# Autodesk Inventor assembly: AK-C-C39-USB-Board-Assembly
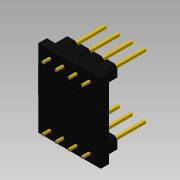
[picture p0: Inventor's stored thumbnail of the model, 180x180]
Saved by Autodesk Inventor 2016 (Build 200138000, 138)
## iProperties
Created: 2016-06-09
Part Number: AK-C-C39-USB-Board-Assembly
Document SubType Name: Assembly
Designer: admin
Author: admin
## Documents named in this file (4)
- E:\Alex\DI-Lambda\parts\v1\AK-C-C39\AK-C-C39-USB-Board-Assembly.iam
- E:\Alex\DI-Lambda\parts\v1\AK-C-C39\Ak-C-C39-USB-board.ipt
- E:\Alex\DI-Lambda\parts\Common\fciconnect-10118194.ipt
- E:\Alex\DI-Lambda\parts\Common\Pin-round-2.54-male.ipt
## Components (10 placed, 3 different names)
1. Ak-C-C39-USB-board:1 — Mate:7, Mate:8, Mate:9, Mate:10, Mate:15, Angle:1, Mate:17
2. fciconnect-10118194:1 — Mate:7, Mate:10
3. Pin-round-2.54-male:1 — Mate:1, Flush:2, Flush:6, Mate:13, Flush:13
4. Pin-round-2.54-male:2 — Mate:1, Mate:2, Flush:3, Flush:5, Flush:6, Mate:8, Mate:16
5. Pin-round-2.54-male:3 — Mate:2, Mate:3, Flush:1, Flush:3, Flush:4, Flush:5
6. Pin-round-2.54-male:4 — Mate:3, Flush:1, Flush:2, Flush:4, Angle:1
7. Pin-round-2.54-male:5 — Flush:7, Flush:10, Mate:4, Mate:17
8. Pin-round-2.54-male:6 — Flush:7, Flush:8, Flush:10, Flush:11, Mate:4, Mate:5, Mate:9
9. Pin-round-2.54-male:7 — Flush:8, Flush:9, Flush:11, Flush:12, Mate:5, Mate:6
10. Pin-round-2.54-male:8 — Flush:9, Flush:12, Mate:6, Mate:12, Flush:13
## Relationships (30: Mate 16, Flush 13, Angle 1)
- Mate:1: Pin-round-2.54-male:1 ↔ Pin-round-2.54-male:2
- Mate:2: Pin-round-2.54-male:2 ↔ Pin-round-2.54-male:3
- Mate:3: Pin-round-2.54-male:3 ↔ Pin-round-2.54-male:4
- Flush:1: Pin-round-2.54-male:3 ↔ Pin-round-2.54-male:4
- Flush:2: Pin-round-2.54-male:1 ↔ Pin-round-2.54-male:4
- Flush:3: Pin-round-2.54-male:2 ↔ Pin-round-2.54-male:3
- Flush:4: Pin-round-2.54-male:3 ↔ Pin-round-2.54-male:4
- Flush:5: Pin-round-2.54-male:2 ↔ Pin-round-2.54-male:3
- Flush:6: Pin-round-2.54-male:1 ↔ Pin-round-2.54-male:2
- Flush:7: Pin-round-2.54-male:5 ↔ Pin-round-2.54-male:6
- Flush:8: Pin-round-2.54-male:6 ↔ Pin-round-2.54-male:7
- Flush:9: Pin-round-2.54-male:7 ↔ Pin-round-2.54-male:8
- Flush:10: Pin-round-2.54-male:5 ↔ Pin-round-2.54-male:6
- Flush:11: Pin-round-2.54-male:6 ↔ Pin-round-2.54-male:7
- Flush:12: Pin-round-2.54-male:7 ↔ Pin-round-2.54-male:8
- Mate:4: Pin-round-2.54-male:5 ↔ Pin-round-2.54-male:6
- Mate:5: Pin-round-2.54-male:6 ↔ Pin-round-2.54-male:7
- Mate:6: Pin-round-2.54-male:7 ↔ Pin-round-2.54-male:8
- Mate:7: Ak-C-C39-USB-board:1 ↔ fciconnect-10118194:1
- Mate:8: Ak-C-C39-USB-board:1 ↔ Pin-round-2.54-male:2
- Mate:9: Ak-C-C39-USB-board:1 ↔ Pin-round-2.54-male:6
- Mate:10: Ak-C-C39-USB-board:1 ↔ fciconnect-10118194:1
- Mate:12: Pin-round-2.54-male:8
- Mate:13: Pin-round-2.54-male:1
- Mate:14 (12 mm)
- Flush:13: Pin-round-2.54-male:1 ↔ Pin-round-2.54-male:8
- Mate:15: Ak-C-C39-USB-board:1
- Mate:16: Pin-round-2.54-male:2
- Angle:1 (0 deg): Ak-C-C39-USB-board:1 ↔ Pin-round-2.54-male:4
- Mate:17 (-1.5 mm): Ak-C-C39-USB-board:1 ↔ Pin-round-2.54-male:5
